# Autodesk Inventor assembly: FrameAssembly
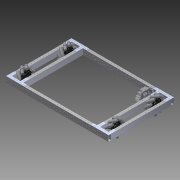
[picture p0: Inventor's stored thumbnail of the model, 180x180]
Saved by Autodesk Inventor 2014 SP1 (Build 180222100, 222)
## iProperties
Created: 2014-01-10
Part Number: FrameAssembly
Document SubType Name: Assembly
Designer: Paul
Author: Paul
## Documents named in this file (10)
- C:\Users\Paul\Documents\Robotics\CAD\Robot\Drivetrain\Drivetrain Assembly\FrameAssembly .iam
- C:\Users\Paul\Documents\Robotics\CAD\Robot\Structure\Frame Assembly\2x1 Tube 21in.ipt
- C:\Users\Paul\Documents\Robotics\CAD\Robot\Structure\Frame Assembly\2x1 Tube 34in.ipt
- C:\Users\Paul\Documents\Robotics\CAD\Robot\Drivetrain\Drivetrain Assembly\Imported Components\Left Mechanum\Left Mechanum.iam
- C:\Users\Paul\Documents\Robotics\CAD\Robot\Drivetrain\Drivetrain Assembly\Imported Components\Right mechanum\Right mechanum.iam
- C:\Users\Paul\Documents\Robotics\CAD\Robot\Structure\Imported Components\T Guesset\T Guesset.ipt
- C:\Users\Paul\Documents\Robotics\CAD\Robot\Drivetrain\Imported Components\Hex Versa Hub\Hex Versa Hub.ipt
- C:\Users\Paul\Documents\Robotics\CAD\Robot\Structure\Imported Components\L Guesset\L Guesset.ipt
- C:\Users\Paul\Documents\Robotics\CAD\Robot\KOP STEP\Drive Base Kit\FIRST Drive Base Long\Parts\Imported Components\Toughbox Mini L-Base.iam\Toughbox Mini L-Base.iam.iam
- Toughbox Mini L-Base.iam
## Components (20 placed, 8 different names)
1. 2x1 Tube 21in:1 — Mate:39, Mate:42, Mate:44, Mate:47, Mate:48, Mate:54, Mate:57, Mate:61, Mate:62
2. 2x1 Tube 21in:2 — Mate:49, Mate:50, Mate:55, Mate:56, Mate:58, Mate:59, Mate:60, Mate:77
3. 2x1 Tube 34in:1 — Mate:41, Mate:49, Mate:53, Mate:54, Flush:1, Mate:74, Mate:75, Mate:76, Mate:84, Mate:85
4. 2x1 Tube 34in:2 — Mate:45, Mate:48, Flush:1, Mate:67, Mate:68, Mate:70, Mate:78, Mate:80, Mate:81
5. Left Mechanum:1 [sub-assembly]
6. Left Mechanum:2 [sub-assembly]
7. Right mechanum:1 [sub-assembly] — Mate:64, Mate:65, Mate:66
8. Right mechanum:2 [sub-assembly]
9. T Guesset:1 — Mate:39, Mate:41, Mate:42, Mate:44
10. T Guesset:4 — Mate:58, Mate:59, Mate:60
11. T Guesset:5 — Mate:50, Mate:53, Mate:55, Mate:56
12. T Guesset:6 — Mate:45, Mate:47, Mate:57, Mate:61, Mate:62
13. Hex Versa Hub:1 — Mate:64, Mate:65, Mate:66
14. 2x1 Tube 21in:3 — Mate:69, Mate:71, Mate:72, Mate:73
15. 2x1 Tube 21in:4 — Mate:79, Mate:82, Mate:83
16. L Guesset:1 — Mate:67, Mate:68, Mate:69, Mate:70, Mate:71, Mate:72, Mate:73
17. L Guesset:2 — Mate:74, Mate:75, Mate:76
18. Toughbox Mini L-Base.iam:1 [sub-assembly] — Mate:77
19. L Guesset:3 — Mate:84, Mate:85
20. L Guesset:4 — Mate:78, Mate:79, Mate:80, Mate:81, Mate:82, Mate:83
## Relationships (42: Mate 41, Flush 1)
- Mate:39: 2x1 Tube 21in:1 ↔ T Guesset:1
- Mate:41: 2x1 Tube 34in:1 ↔ T Guesset:1
- Mate:42: 2x1 Tube 21in:1 ↔ T Guesset:1
- Mate:44: 2x1 Tube 21in:1 ↔ T Guesset:1
- Mate:45: 2x1 Tube 34in:2 ↔ T Guesset:6
- Mate:47: 2x1 Tube 21in:1 ↔ T Guesset:6
- Mate:48: 2x1 Tube 21in:1 ↔ 2x1 Tube 34in:2
- Mate:49: 2x1 Tube 21in:2 ↔ 2x1 Tube 34in:1
- Mate:50: 2x1 Tube 21in:2 ↔ T Guesset:5
- Mate:53: 2x1 Tube 34in:1 ↔ T Guesset:5
- Mate:54: 2x1 Tube 21in:1 ↔ 2x1 Tube 34in:1
- Mate:55: 2x1 Tube 21in:2 ↔ T Guesset:5
- Mate:56: 2x1 Tube 21in:2 ↔ T Guesset:5
- Flush:1: 2x1 Tube 34in:1 ↔ 2x1 Tube 34in:2
- Mate:57: 2x1 Tube 21in:1 ↔ T Guesset:6
- Mate:58: 2x1 Tube 21in:2 ↔ T Guesset:4
- Mate:59: 2x1 Tube 21in:2 ↔ T Guesset:4
- Mate:60: 2x1 Tube 21in:2 ↔ T Guesset:4
- Mate:61: 2x1 Tube 21in:1 ↔ T Guesset:6
- Mate:62: 2x1 Tube 21in:1 ↔ T Guesset:6
- Mate:64: Right mechanum:1 ↔ Hex Versa Hub:1
- Mate:65: Right mechanum:1 ↔ Hex Versa Hub:1
- Mate:66: Right mechanum:1 ↔ Hex Versa Hub:1
- Mate:67: 2x1 Tube 34in:2 ↔ L Guesset:1
- Mate:68: 2x1 Tube 34in:2 ↔ L Guesset:1
- Mate:69: 2x1 Tube 21in:3 ↔ L Guesset:1
- Mate:70: 2x1 Tube 34in:2 ↔ L Guesset:1
- Mate:71: 2x1 Tube 21in:3 ↔ L Guesset:1
- Mate:72: 2x1 Tube 21in:3 ↔ L Guesset:1
- Mate:73: 2x1 Tube 21in:3 ↔ L Guesset:1
- Mate:74: 2x1 Tube 34in:1 ↔ L Guesset:2
- Mate:75: 2x1 Tube 34in:1 ↔ L Guesset:2
- Mate:76: 2x1 Tube 34in:1 ↔ L Guesset:2
- Mate:77: 2x1 Tube 21in:2 ↔ Toughbox Mini L-Base.iam:1
- Mate:78: 2x1 Tube 34in:2 ↔ L Guesset:4
- Mate:79: 2x1 Tube 21in:4 ↔ L Guesset:4
- Mate:80: 2x1 Tube 34in:2 ↔ L Guesset:4
- Mate:81: 2x1 Tube 34in:2 ↔ L Guesset:4
- Mate:82: 2x1 Tube 21in:4 ↔ L Guesset:4
- Mate:83: 2x1 Tube 21in:4 ↔ L Guesset:4
- Mate:84: 2x1 Tube 34in:1 ↔ L Guesset:3
- Mate:85: 2x1 Tube 34in:1 ↔ L Guesset:3
